# Autodesk Inventor assembly: søjle+vange
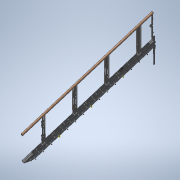
[picture p0: Inventor's stored thumbnail of the model, 180x180]
Saved by Autodesk Inventor 2020.1 (Build 241239000, 239)
## iProperties
Created: 2019-09-25
Part Number: søjle+vange
Document SubType Name: Assembly
Designer: Kristoffer Ek
Mass: 165952 g
Surface Area: 103178 cm^2
Volume: 42097.6 cm^3
Density: 3.94208 g/cm^3
Description: Beplantet bæredygtig trappe
Engineer: Kristoffer Ek
Authority: Loppen
Author: Kristoffer Ek
Title: Beplantet bæredygtig trappe
## Documents named in this file (36)
- Y:\trappe\søjle+vange.iam
- Y:\trappe\modul top.iam
- Y:\trappe\søjle\stilladssøjle.iam
- Y:\trappe\modul.iam
- Y:\trappe\modul bund.iam
- Y:\trappe\håndfang\træhåndfang.ipt
- Y:\trappe\hegn\hegnspæl.iam
- Y:\trappe\hegn\hegnspæl omvendt.iam
- Y:\trappe\søjle+vange\Design Accelerator\Bolted Connection1.iam
- Y:\trappe\søjle+vange\Design Accelerator\Bolted Connection2.iam
- Y:\trappe\søjle+vange\Design Accelerator\Bolted Connection3.iam
- Y:\trappe\søjle+vange\Design Accelerator\Bolted Connection4.iam
- Y:\trappe\søjle+vange\Design Accelerator\Bolted Connection5.iam
- Y:\trappe\søjle+vange\Design Accelerator\Bolted Connection6.iam
- Y:\trappe\søjle+vange\Design Accelerator\Bolted Connection7.iam
- Y:\trappe\søjle+vange\Design Accelerator\Bolted Connection8.iam
- Y:\trappe\søjle+vange\Design Accelerator\Bolted Connection9.iam
- Y:\trappe\søjle+vange\Design Accelerator\Bolted Connection10.iam
- Y:\trappe\søjle+vange\Design Accelerator\Bolted Connection11.iam
- Y:\trappe\søjle+vange\Design Accelerator\Bolted Connection12.iam
- Y:\trappe\søjle+vange\Design Accelerator\Bolted Connection13.iam
- Y:\trappe\søjle+vange\Design Accelerator\Bolted Connection14.iam
- Y:\trappe\søjle+vange\Design Accelerator\Bolted Connection15.iam
- Y:\trappe\søjle+vange\Design Accelerator\Bolted Connection16.iam
- Y:\trappe\søjle+vange\Design Accelerator\Bolted Connection17.iam
- Y:\trappe\søjle+vange\Design Accelerator\Bolted Connection18.iam
- Y:\trappe\søjle+vange\Design Accelerator\Bolted Connection19.iam
- Y:\trappe\søjle+vange\Design Accelerator\Bolted Connection20.iam
- Y:\trappe\søjle+vange\Design Accelerator\Bolted Connection21.iam
- Y:\trappe\søjle+vange\Design Accelerator\Bolted Connection22.iam
- Y:\trappe\søjle+vange\Design Accelerator\Bolted Connection23.iam
- Y:\trappe\søjle+vange\Design Accelerator\Bolted Connection24.iam
- Y:\trappe\hegn\hegnspæl, oppe, top.iam
- hegnspæl.iam
- Y:\trappe\håndfang\led-liste.ipt
- Y:\trappe\håndfang\acryl-difuseringsplader.ipt
## Components (43 placed, 10 different names)
1. stilladssøjle:2 [sub-assembly] — Mate:3, Mate:4, øre, Mate:14, Tangent:4
2. modul top:1 [sub-assembly] — Mate:3, Mate:4, øre, Flush:1, Flush:3, Mate:6, Mate:10, Mate:11, Flush:10, Tangent:1, Mate:13, Mate:34, Tangent:11, Mate:73, Mate:76, Mate:77, Mate:94, Mate:96, Mate:98, Mate:100, Mate:102, Mate:104, Mate:106
3. modul:1 [sub-assembly] — Flush:1, Flush:2, Flush:3, Flush:4, Mate:6, Mate:7, Flush:13, Mate:15, Tangent:5, Mate:33, Mate:48, Mate:50, Mate:74, Tangent:12, Mate:75, Mate:93, Mate:95, Mate:97, Mate:99, Mate:101, Mate:103, Mate:105, Mate:110, Mate:112
4. modul:2 [sub-assembly] — Flush:2, Flush:4, Mate:7, Flush:5, Flush:6, Flush:7, Mate:8, Flush:15, Mate:16, Mate:17, Tangent:7, Mate:39, Mate:40, Mate:41, Mate:42, Mate:43, Mate:44, Mate:45, Mate:46, Mate:47, Mate:49, Mate:56, Mate:58, Mate:64, Mate:66, Tangent:9, Mate:71, Mate:108, Mate:109, Mate:111, Mate:114, Mate:116, Mate:118
5. modul bund:1 [sub-assembly] — Flush:5, Flush:6, Flush:7, Mate:8, Mate:18, Mate:55, Mate:57, Mate:63, Mate:65, Tangent:10, Mate:72, Mate:107, Mate:113, Mate:115, Mate:117
6. træhåndfang:1 — Mate:10, Mate:76, Mate:77, Mate:78, Mate:79, Mate:80, Mate:81, Mate:82, Mate:83, Mate:84, Mate:85, Mate:86, Mate:87, Mate:88, Mate:92
7. hegnspæl:1 [sub-assembly] — Mate:11, Flush:10, Tangent:1
8. hegnspæl omvendt:1 [sub-assembly] — Mate:74, Tangent:12, Mate:75
9. hegnspæl:2 [sub-assembly] — Flush:13, Mate:15, Tangent:5
10. hegnspæl omvendt:2 [sub-assembly] — Mate:16, Tangent:9, Mate:71
11. hegnspæl:3 [sub-assembly] — Flush:15, Mate:17, Tangent:7
12. hegnspæl omvendt:3 [sub-assembly] — Mate:18, Tangent:10, Mate:72
13. hegnspæl:4 [sub-assembly] — Mate:14, Tangent:4
14. hegnspæl omvendt:4 [sub-assembly] — Mate:13, Tangent:11, Mate:73
15. Bolted Connection:1 [sub-assembly] — Mate:93, Mate:94
16. Bolted Connection:2 [sub-assembly] — Mate:95, Mate:96
17. Bolted Connection:3 [sub-assembly] — Mate:97, Mate:98
18. Bolted Connection:4 [sub-assembly] — Mate:99, Mate:100
19. Bolted Connection:5 [sub-assembly] — Mate:101, Mate:102
20. Bolted Connection:6 [sub-assembly] — Mate:33, Mate:34
21. Bolted Connection:7 [sub-assembly] — Mate:103, Mate:104
22. Bolted Connection:8 [sub-assembly] — Mate:105, Mate:106
23. Bolted Connection:9 [sub-assembly] — Mate:39, Mate:40
24. Bolted Connection:10 [sub-assembly] — Mate:41, Mate:42
25. Bolted Connection:11 [sub-assembly] — Mate:43, Mate:44
26. Bolted Connection:12 [sub-assembly] — Mate:45, Mate:46
27. Bolted Connection:13 [sub-assembly] — Mate:47, Mate:48
28. Bolted Connection:14 [sub-assembly] — Mate:49, Mate:50
29. Bolted Connection:15 [sub-assembly] — Mate:109, Mate:110
30. Bolted Connection:16 [sub-assembly] — Mate:111, Mate:112
31. Bolted Connection:17 [sub-assembly] — Mate:55, Mate:56
32. Bolted Connection:18 [sub-assembly] — Mate:57, Mate:58
33. Bolted Connection:19 [sub-assembly] — Mate:117, Mate:118
34. Bolted Connection:20 [sub-assembly] — Mate:115, Mate:116
35. Bolted Connection:21 [sub-assembly] — Mate:63, Mate:64
36. Bolted Connection:22 [sub-assembly] — Mate:65, Mate:66
37. Bolted Connection:23 [sub-assembly] — Mate:113, Mate:114
38. Bolted Connection:24 [sub-assembly] — Mate:107, Mate:108
39. led-liste:1 — Mate:78, Mate:79, Mate:80
40. acryl-difuseringsplader:1 — Mate:81, Mate:85, Mate:89, Mate:92
41. acryl-difuseringsplader:2 — Mate:82, Mate:86, Mate:89, Mate:90
42. acryl-difuseringsplader:3 — Mate:83, Mate:87, Mate:90, Mate:91
43. acryl-difuseringsplader:4 — Mate:84, Mate:88, Mate:91
## Relationships (103: Mate 85, Flush 10, Tangent 8)
- [Mate]: stilladssøjle:2 ↔ modul top:1
- Mate:3: stilladssøjle:2 ↔ modul top:1
- Mate:4: stilladssøjle:2 ↔ modul top:1
- øre [Mate]: stilladssøjle:2 ↔ modul top:1
- Flush:1: modul top:1 ↔ modul:1
- Flush:2: modul:1 ↔ modul:2
- Flush:3: modul top:1 ↔ modul:1
- Flush:4: modul:1 ↔ modul:2
- Mate:6 (2 mm): modul top:1 ↔ modul:1
- Mate:7 (2 mm): modul:1 ↔ modul:2
- Flush:5: modul:2 ↔ modul bund:1
- Flush:6: modul:2 ↔ modul bund:1
- Flush:7: modul:2 ↔ modul bund:1
- Mate:8 (2 mm): modul:2 ↔ modul bund:1
- Mate:10: modul top:1 ↔ træhåndfang:1
- Mate:11: modul top:1 ↔ hegnspæl:1
- Flush:10: modul top:1 ↔ hegnspæl:1
- Tangent:1: modul top:1 ↔ hegnspæl:1
- Mate:13: modul top:1 ↔ hegnspæl omvendt:4
- Mate:14: stilladssøjle:2 ↔ hegnspæl:4
- Tangent:4: stilladssøjle:2 ↔ hegnspæl:4
- Flush:13: modul:1 ↔ hegnspæl:2
- Flush:15: modul:2 ↔ hegnspæl:3
- Mate:15: modul:1 ↔ hegnspæl:2
- Tangent:5: modul:1 ↔ hegnspæl:2
- Mate:16: modul:2 ↔ hegnspæl omvendt:2
- Mate:17: modul:2 ↔ hegnspæl:3
- Mate:18: modul bund:1 ↔ hegnspæl omvendt:3
- Tangent:7: modul:2 ↔ hegnspæl:3
- Mate:33: modul:1 ↔ Bolted Connection:6
- Mate:34: modul top:1 ↔ Bolted Connection:6
- Mate:39: modul:2 ↔ Bolted Connection:9
- Mate:40: modul:2 ↔ Bolted Connection:9
- Mate:41: modul:2 ↔ Bolted Connection:10
- Mate:42: modul:2 ↔ Bolted Connection:10
- Mate:43: modul:2 ↔ Bolted Connection:11
- Mate:44: modul:2 ↔ Bolted Connection:11
- Mate:45: modul:2 ↔ Bolted Connection:12
- Mate:46: modul:2 ↔ Bolted Connection:12
- Mate:47: modul:2 ↔ Bolted Connection:13
- Mate:48: modul:1 ↔ Bolted Connection:13
- Mate:49: modul:2 ↔ Bolted Connection:14
- Mate:50: modul:1 ↔ Bolted Connection:14
- Mate:55: modul bund:1 ↔ Bolted Connection:17
- Mate:56: modul:2 ↔ Bolted Connection:17
- Mate:57: modul bund:1 ↔ Bolted Connection:18
- Mate:58: modul:2 ↔ Bolted Connection:18
- Mate:63: modul bund:1 ↔ Bolted Connection:21
- Mate:64: modul:2 ↔ Bolted Connection:21
- Mate:65: modul bund:1 ↔ Bolted Connection:22
- Mate:66: modul:2 ↔ Bolted Connection:22
- Tangent:9: modul:2 ↔ hegnspæl omvendt:2
- Mate:71: modul:2 ↔ hegnspæl omvendt:2
- Tangent:10: modul bund:1 ↔ hegnspæl omvendt:3
- Mate:72: modul bund:1 ↔ hegnspæl omvendt:3
- Tangent:11: modul top:1 ↔ hegnspæl omvendt:4
- Mate:73: modul top:1 ↔ hegnspæl omvendt:4
- Mate:74: modul:1 ↔ hegnspæl omvendt:1
- Tangent:12: modul:1 ↔ hegnspæl omvendt:1
- Mate:75: modul:1 ↔ hegnspæl omvendt:1
- Mate:76: modul top:1 ↔ træhåndfang:1
- Mate:77 (1.5 mm): modul top:1 ↔ træhåndfang:1
- Mate:78: træhåndfang:1 ↔ led-liste:1
- Mate:79: træhåndfang:1 ↔ led-liste:1
- Mate:80: træhåndfang:1 ↔ led-liste:1
- Mate:81: træhåndfang:1 ↔ acryl-difuseringsplader:1
- Mate:82: træhåndfang:1 ↔ acryl-difuseringsplader:2
- Mate:83: træhåndfang:1 ↔ acryl-difuseringsplader:3
- Mate:84: træhåndfang:1 ↔ acryl-difuseringsplader:4
- Mate:85: træhåndfang:1 ↔ acryl-difuseringsplader:1
- Mate:86: træhåndfang:1 ↔ acryl-difuseringsplader:2
- Mate:87: træhåndfang:1 ↔ acryl-difuseringsplader:3
- Mate:88: træhåndfang:1 ↔ acryl-difuseringsplader:4
- Mate:89 (1 mm): acryl-difuseringsplader:1 ↔ acryl-difuseringsplader:2
- Mate:90 (1 mm): acryl-difuseringsplader:2 ↔ acryl-difuseringsplader:3
- Mate:91 (1 mm): acryl-difuseringsplader:3 ↔ acryl-difuseringsplader:4
- Mate:92 (5 mm): træhåndfang:1 ↔ acryl-difuseringsplader:1
- Mate:93: modul:1 ↔ Bolted Connection:1
- Mate:94: modul top:1 ↔ Bolted Connection:1
- Mate:95: modul:1 ↔ Bolted Connection:2
- Mate:96: modul top:1 ↔ Bolted Connection:2
- Mate:97: modul:1 ↔ Bolted Connection:3
- Mate:98: modul top:1 ↔ Bolted Connection:3
- Mate:99: modul:1 ↔ Bolted Connection:4
- Mate:100: modul top:1 ↔ Bolted Connection:4
- Mate:101: modul:1 ↔ Bolted Connection:5
- Mate:102: modul top:1 ↔ Bolted Connection:5
- Mate:103: modul:1 ↔ Bolted Connection:7
- Mate:104: modul top:1 ↔ Bolted Connection:7
- Mate:105: modul:1 ↔ Bolted Connection:8
- Mate:106: modul top:1 ↔ Bolted Connection:8
- Mate:107: modul bund:1 ↔ Bolted Connection:24
- Mate:108: modul:2 ↔ Bolted Connection:24
- Mate:109: modul:2 ↔ Bolted Connection:15
- Mate:110: modul:1 ↔ Bolted Connection:15
- Mate:111: modul:2 ↔ Bolted Connection:16
- Mate:112: modul:1 ↔ Bolted Connection:16
- Mate:113: modul bund:1 ↔ Bolted Connection:23
- Mate:114: modul:2 ↔ Bolted Connection:23
- Mate:115: modul bund:1 ↔ Bolted Connection:20
- Mate:116: modul:2 ↔ Bolted Connection:20
- Mate:117: modul bund:1 ↔ Bolted Connection:19
- Mate:118: modul:2 ↔ Bolted Connection:19
